# Autodesk Inventor assembly: frame assembly 2
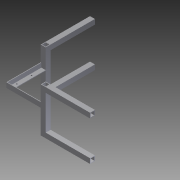
[picture p0: Inventor's stored thumbnail of the model, 180x180]
Saved by Autodesk Inventor 2012 (Build 160160000, 160)
## iProperties
Created: 2013-01-04
Part Number: frame assembly 2
Document SubType Name: Assembly
Designer: Bryce
Author: Bryce
## Documents named in this file (4)
- C:\Users\Bryce\Dropbox\Inventor Design Project Files\Independent Swerves\Inventor 2012\frame assembly 2.iam
- C:\Users\Bryce\Dropbox\Inventor Design Project Files\Independent Swerves\Inventor 2012\left frame peace 2.ipt
- C:\Users\Bryce\Dropbox\Inventor Design Project Files\Independent Swerves\Inventor 2012\right frame peace 2.ipt
- C:\Users\Bryce\Dropbox\Inventor Design Project Files\Independent Swerves\Inventor 2012\vertical frame piece.ipt
## Components (8 placed, 3 different names)
1. left frame peace 2:1 — Mate:1, Flush:1, Mate:2, Flush:4, Mate:4, Flush:13
2. right frame peace 2:1 — Mate:1, Flush:1, Mate:2, Mate:3, Flush:2
3. vertical frame piece:1 — Mate:3, Flush:2, Flush:3, Mate:5, Flush:5, Flush:6, Flush:7, Flush:8, Mate:6
4. vertical frame piece:2 — Flush:3, Flush:4, Mate:4, Mate:7, Flush:9, Flush:10, Mate:8, Flush:11, Flush:12, Flush:13
5. vertical frame piece:3 — Mate:8, Flush:11, Flush:12
6. vertical frame piece:4 — Mate:5, Flush:5, Flush:6
7. vertical frame piece:5 — Mate:7, Flush:9, Flush:10
8. vertical frame piece:6 — Flush:7, Flush:8, Mate:6
## Relationships (21: Flush 13, Mate 8)
- Mate:1: left frame peace 2:1 ↔ right frame peace 2:1
- Flush:1: left frame peace 2:1 ↔ right frame peace 2:1
- Mate:2: left frame peace 2:1 ↔ right frame peace 2:1
- Mate:3: right frame peace 2:1 ↔ vertical frame piece:1
- Flush:2: right frame peace 2:1 ↔ vertical frame piece:1
- Flush:3: vertical frame piece:1 ↔ vertical frame piece:2
- Flush:4: left frame peace 2:1 ↔ vertical frame piece:2
- Mate:4: left frame peace 2:1 ↔ vertical frame piece:2
- Mate:5: vertical frame piece:1 ↔ vertical frame piece:4
- Flush:5: vertical frame piece:1 ↔ vertical frame piece:4
- Flush:6: vertical frame piece:1 ↔ vertical frame piece:4
- Flush:7: vertical frame piece:1 ↔ vertical frame piece:6
- Flush:8: vertical frame piece:1 ↔ vertical frame piece:6
- Mate:6: vertical frame piece:1 ↔ vertical frame piece:6
- Mate:7: vertical frame piece:2 ↔ vertical frame piece:5
- Flush:9: vertical frame piece:2 ↔ vertical frame piece:5
- Flush:10: vertical frame piece:2 ↔ vertical frame piece:5
- Mate:8: vertical frame piece:2 ↔ vertical frame piece:3
- Flush:11: vertical frame piece:2 ↔ vertical frame piece:3
- Flush:12: vertical frame piece:2 ↔ vertical frame piece:3
- Flush:13 (101.6 mm): left frame peace 2:1 ↔ vertical frame piece:2
